# Autodesk Inventor assembly: arms assembly for plow
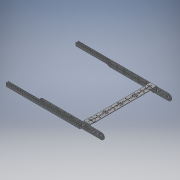
[picture p0: Inventor's stored thumbnail of the model, 180x180]
Saved by Autodesk Inventor 2016 (Build 200138000, 138)
## iProperties
Created: 2015-10-24
Part Number: arms assembly for plow
Document SubType Name: Assembly
Designer: Delta
Author: Delta
## Documents named in this file (4)
- C:\Robotics\2015-16_CAD\custom cad parts\arms assembly for plow.iam
- C:\Robotics\2015-16_CAD\COTSParts\Tetrix\Pitsco Education-739271.iam
- C:\Robotics\2015-16_CAD\COTSParts\Tetrix\Tetrix bracket - angle.ipt
- C:\Robotics\2015-16_CAD\COTSParts\Actobotics\585 parts\585398.ipt
## Components (7 placed, 3 different names)
1. Pitsco Education-739271:1 [sub-assembly] — Insert:1, Insert:2, Insert:3, Insert:4
2. Pitsco Education-739271:2 [sub-assembly] — Insert:5, Insert:6, Mate:2
3. Pitsco Education-739271:3 [sub-assembly] — Insert:7, Insert:8
4. Tetrix bracket - angle:1 — Insert:1, Insert:2, Insert:7, Insert:8
5. Tetrix bracket - angle:2 — Insert:3, Insert:4, Insert:5, Insert:6
6. 585398:1 — Mate:2
7. 585398:2
## Relationships (9: Insert 8, Mate 1)
- Insert:1: Pitsco Education-739271:1 ↔ Tetrix bracket - angle:1
- Insert:2: Pitsco Education-739271:1 ↔ Tetrix bracket - angle:1
- Insert:3: Pitsco Education-739271:1 ↔ Tetrix bracket - angle:2
- Insert:4: Pitsco Education-739271:1 ↔ Tetrix bracket - angle:2
- Insert:5: Pitsco Education-739271:2 ↔ Tetrix bracket - angle:2
- Insert:6: Pitsco Education-739271:2 ↔ Tetrix bracket - angle:2
- Insert:7: Pitsco Education-739271:3 ↔ Tetrix bracket - angle:1
- Insert:8: Pitsco Education-739271:3 ↔ Tetrix bracket - angle:1
- Mate:2: Pitsco Education-739271:2 ↔ 585398:1
